# Autodesk Inventor assembly: body_8d_1
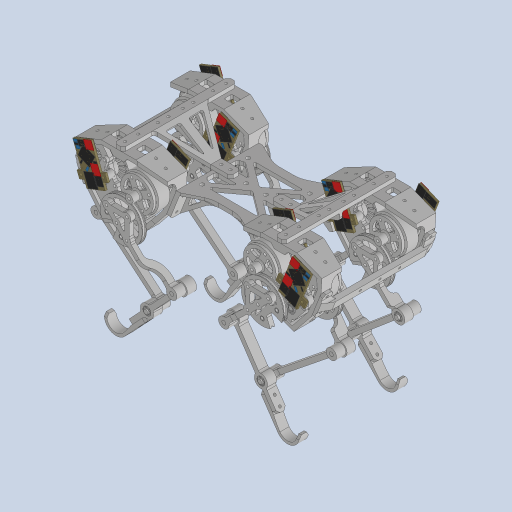
[picture p0: Inventor's stored thumbnail of the model, 512x512]
Saved by Autodesk Inventor 2023 (Build 270158000, 158)
## iProperties
Created: 2021-03-13
Part Number: body_8d_1
Document SubType Name: Assembly
Designer: Shuang Peng
Author: Shuang Peng
## Documents named in this file (6)
- D:\projects-3\biped_tiny\hardware\body_8d_1.iam
- D:\projects-3\biped_tiny\hardware\leg_2d_1.iam
- D:\projects-3\biped_tiny\hardware\leg_1_2d_MIR.iam
- D:\projects-3\biped_tiny\hardware\body_linker_1_8d.ipt
- D:\projects-3\biped_tiny\hardware\body_linker_2_8d.ipt
- D:\projects-3\biped_tiny\hardware\en_shell_1.ipt
## Components (9 placed, 5 different names)
1. leg_2d_1:1 [sub-assembly] — Flush:1, Flush:2, Flush:3, Mate:1, Flush:4, Flush:7, Flush:8
2. leg_1_2d_MIR:1 [sub-assembly] — Flush:3, Mate:1, Flush:4, Mate:3, Flush:13
3. leg_2d_1:2 [sub-assembly] — Mate:3, Symmetry:1, Flush:10, Insert:7
4. leg_1_2d_MIR:2 [sub-assembly] — Flush:7, Flush:8, Flush:9, Symmetry:1, Insert:1, Insert:6
5. body_linker_1_8d:1 — Flush:9, Flush:11, Flush:12, Insert:1, Insert:2, Insert:3, Insert:4, Insert:5
6. body_linker_2_8d:1 — Flush:10, Flush:11, Flush:12, Insert:2, Insert:3
7. body_linker_2_8d:2 — Insert:4, Insert:5
8. en_shell_1:1 — Flush:13
9. en_shell_1:2 — Insert:6, Insert:7
## Relationships (24: Flush 13, Insert 7, Mate 3, Symmetry 1)
- Flush:1: leg_2d_1:1
- Flush:2: leg_2d_1:1
- Flush:3: leg_2d_1:1 ↔ leg_1_2d_MIR:1
- Mate:1 (-87 mm): leg_2d_1:1 ↔ leg_1_2d_MIR:1
- Flush:4: leg_2d_1:1 ↔ leg_1_2d_MIR:1
- [Flush]: leg_2d_1:2 ↔ leg_1_2d_MIR:2
- [Mate] (-87 mm): leg_2d_1:2 ↔ leg_1_2d_MIR:2
- [Flush]: leg_2d_1:2 ↔ leg_1_2d_MIR:2
- Flush:7: leg_2d_1:1 ↔ leg_1_2d_MIR:2
- Flush:8: leg_2d_1:1 ↔ leg_1_2d_MIR:2
- Mate:3 (110 mm): leg_1_2d_MIR:1 ↔ leg_2d_1:2
- Flush:9: leg_1_2d_MIR:2 ↔ body_linker_1_8d:1
- Symmetry:1: leg_2d_1:2 ↔ leg_1_2d_MIR:2
- Flush:10: leg_2d_1:2 ↔ body_linker_2_8d:1
- Flush:11: body_linker_1_8d:1 ↔ body_linker_2_8d:1
- Flush:12: body_linker_1_8d:1 ↔ body_linker_2_8d:1
- Insert:1: leg_1_2d_MIR:2 ↔ body_linker_1_8d:1
- Insert:2: body_linker_1_8d:1 ↔ body_linker_2_8d:1
- Insert:3: body_linker_1_8d:1 ↔ body_linker_2_8d:1
- Insert:4: body_linker_1_8d:1 ↔ body_linker_2_8d:2
- Insert:5: body_linker_1_8d:1 ↔ body_linker_2_8d:2
- Flush:13: leg_1_2d_MIR:1 ↔ en_shell_1:1
- Insert:6: leg_1_2d_MIR:2 ↔ en_shell_1:2
- Insert:7: leg_2d_1:2 ↔ en_shell_1:2
## Named parameters: d6_d3 = 0 mm, d7_d4 = -87 mm, d8_d5 = 0 mm
